# Autodesk Inventor assembly: Robot
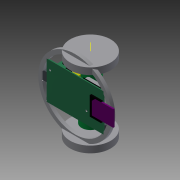
[picture p0: Inventor's stored thumbnail of the model, 180x180]
Saved by Autodesk Inventor 2014 (Build 180170000, 170)
## iProperties
Created: 2013-05-24
Part Number: Robot
Document SubType Name: Assembly
Designer: hartmann
Author: hartmann
## Documents named in this file (6)
- C:\Users\Felix\Desktop\Beep\Hardware\Robot\Robot.iam
- C:\Users\Felix\Desktop\Beep\Hardware\RaspberryPi\RaspberryPi.iam
- C:\Users\Felix\Desktop\Beep\Hardware\Robot\frame.ipt
- C:\Users\Felix\Desktop\Beep\Hardware\Robot\BaneBots2375.ipt
- C:\Users\Felix\Desktop\Beep\Hardware\Model2\motor.ipt
- C:\Users\Felix\Desktop\Beep\Hardware\Z132053\Z.iam
## Components (8 placed, 5 different names)
1. RaspberryPi:1 [sub-assembly] — Fluchtend:1
2. frame:1 — Fluchtend:1
3. BaneBots2375:1 — Passend:1, Passend:2, Mate:5
4. BaneBots2375:2 — Passend:1, Passend:3, Mate:6
5. motor:1 — Passend:2, Passend:4
6. motor:2 — Passend:3, Passend:4
7. Z:1 [sub-assembly] — Mate:5
8. Z:2 [sub-assembly] — Mate:6
## Relationships (7: Mate 6, Flush 1)
- Fluchtend:1 [Flush]: RaspberryPi:1 ↔ frame:1
- Passend:1 [Mate]: BaneBots2375:1 ↔ BaneBots2375:2
- Passend:2 [Mate]: BaneBots2375:1 ↔ motor:1
- Passend:3 [Mate]: BaneBots2375:2 ↔ motor:2
- Passend:4 [Mate]: motor:1 ↔ motor:2
- Mate:5: BaneBots2375:1 ↔ Z:1
- Mate:6: BaneBots2375:2 ↔ Z:2
